# Autodesk Inventor assembly: My Room
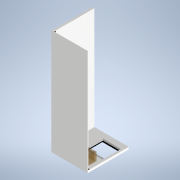
[picture p0: Inventor's stored thumbnail of the model, 180x180]
Saved by Autodesk Inventor 2020 (Build 240168000, 168)
## iProperties
Created: 2021-01-02
Part Number: My Room
Document SubType Name: Assembly
Designer: frost
Author: frost
## Documents named in this file (3)
- C:\Users\frost\OneDrive\Desktop\My Room\My Room.iam
- C:\Users\frost\OneDrive\Desktop\My Room\Room Layout.ipt
- C:\Users\frost\OneDrive\Desktop\My Room\Work Table.ipt
## Components (3 placed, 2 different names)
1. Room Layout:1 — Mate:1, Mate:2, Mate:3, Mate:4
2. Work Table:1 — Mate:1, Mate:2
3. Work Table:2 — Mate:3, Mate:4
## Relationships (4: Mate 4)
- Mate:1: Room Layout:1 ↔ Work Table:1
- Mate:2: Room Layout:1 ↔ Work Table:1
- Mate:3: Room Layout:1 ↔ Work Table:2
- Mate:4: Room Layout:1 ↔ Work Table:2
